# Autodesk Inventor assembly: SansRotor
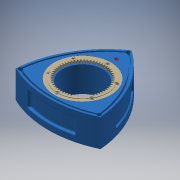
[picture p0: Inventor's stored thumbnail of the model, 180x180]
Saved by Autodesk Inventor 2019 (Build 230136000, 136)
## iProperties
Created: 2019-05-06
Part Number: SansRotor
Document SubType Name: Assembly
Designer: forev
Author: forev
## Documents named in this file (4)
- S:\Git_Repositories\Inventor_Projects\Wankel_Engine\SansRotor.iam
- S:\Univer\( G A C  ) Grafica asistată de calculator\Fișiere necesare\Fisiere necesare teme Inventor\6 - Wankel\Rotor.ipt
- S:\Univer\( G A C  ) Grafica asistată de calculator\Fișiere necesare\Fisiere necesare teme Inventor\6 - Wankel\Roata.ipt
- S:\Git_Repositories\Inventor_Projects\Wankel_Engine\SubAns-M4.iam
## Components (3 placed, 3 different names)
1. Rotor:1 — Mate:1, Mate:2, Mate:3, Mate:4, Mate:5, Angle:1
2. Roata:1 — Mate:4, Mate:5, Angle:1
3. SubAns-M4:1 [sub-assembly]
## Relationships (13: Mate 12, Angle 1)
- Mate:1: Rotor:1
- Mate:2: Rotor:1
- Mate:3: Rotor:1
- Mate:4: Rotor:1 ↔ Roata:1
- Mate:5: Rotor:1 ↔ Roata:1
- Angle:1 (0 deg): Rotor:1 ↔ Roata:1
- [Mate]: Rotor:1 ↔ SubAns-M4:1
- [Mate]: Rotor:1 ↔ SubAns-M4:1
- [Mate]: Rotor:1 ↔ SubAns-M4:1
- [Mate]: Rotor:1 ↔ SubAns-M4:1
- [Mate]: Rotor:1 ↔ SubAns-M4:1
- [Mate]: Rotor:1 ↔ SubAns-M4:1
- [Mate]: Rotor:1 ↔ SubAns-M4:1
